# Autodesk Inventor assembly: HBLFSNF5-SEC_b
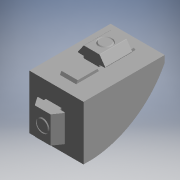
[picture p0: Inventor's stored thumbnail of the model, 180x180]
Saved by Autodesk Inventor 2017.3 (Build 213256000, 256)
## iProperties
Category: PARTsolutions
Company: MISUMI
Part Number: HBLFSNF5-SEC_b
Catalog Web Link: www.cadenas.de
Description: hblfsnf8_blacket-Tabbed Brackets - 1 Slots - HFS5 Series (Aluminum Extrusions 20, 25, 40 Square) - Reversal Tabbed Brackets (Depth 20mm)
Vendor: MISUMI
Document SubType Name: Assembly
Designer: partserver
Manufacturer: MISUMI
Mass: 6.66509 g
Surface Area: 56.4365 cm^2
Volume: 6.66509 cm^3
Density: 1 g/cm^3
Title: HBLFSNF5-SEC
Author: Cadenas PARTsolutions
Comments: Tabbed Brackets - 1 Slots - HFS5 Series (Aluminum Extrusions 20, 25, 40 Square) - Reversal Tabbed Brackets (Depth 20mm)
PSOL_IDENT_0: {$CADENAS_DATA\23d-libs\misumi\metric\38_al_extrusions_blackets\5\hblfsnf5_asmtab.prj},199 {VTYP=3D}
PSOL_IDENT_1: ,{STYP=ASSTAB},{NB=HBLFSNF5-SEC_b},{LINA=HBLFSNF5-SEC},{NN=hblfsnf8_blacket},{DATE=09.09.2019 15:28:
PSOL_IDENT_2: 10},{GEOMDATE=18.03.2016 03:17:17},{VERSION=},{LINEID=10},{WBVAR=ALT1,ALT2},{WBNUMERIC=}  {NB=HBLFSN
PSOL_IDENT_3: F5-SEC_b},{LINA=HBLFSNF5-SEC},{KT=DUMMY},{PN=HBLFSNF5-SEC},{TYPE=HBLFSNF5},{AS=HCBST5-12},{ASQ=2},{A
PSOL_IDENT_4: TN=HNTT5-5},{ATNQ=2},{ALT1=},{ALT2=-SEC},{ALT2ALG= '' , 'w/o Applicable Screws and Nuts Set' , '-SET'
PSOL_IDENT_5: , 'with SET (Applicable Screws and Nuts Set)' , '-SST' , 'with SST (Applicable Screws and Nuts Set(
PSOL_IDENT_6: Stainless Steel))' , '-SEU' , 'with SEU (Applicable Screws and Nuts Set(Pre-Assembly Insertion Sprin
PSOL_IDENT_7: g Nuts))' , '-SSU' , 'with SSU (Applicable Screws and Nuts Set(Pre-Assembly Insertion Spring Nuts St
PSOL_IDENT_8: ainless Steel))'  , '-SEP' , 'with SEP (Applicable Screws and Nuts Set(Post-Assembly Insertion Sprin
PSOL_IDENT_9: g Nuts))' , '-SSP' , 'with SSP (Applicable Screws and Nuts Set(Post-Assembly Insertion Spring Nuts S
PSOL_IDENT_10: tainless Steel))', '-SEC' , 'with SEC (Applicable Screws and Nuts Set(Washer Integrated Screws and N
PSOL_IDENT_11: uts))' },{SMAT=1010 Carbon Steel Equivalent},{SALT2=3},{NALT2=1},{M=5},{PPATH=hblfsnf5/hblfsnf5_asmt
PSOL_IDENT_12: pl.prj}
NB: HBLFSNF5-SEC_b
NN: hblfsnf8_blacket
NT: Tabbed Brackets - 1 Slots - HFS5 Series (Aluminum Extrusions 20, 25, 40 Square) - Reversal Tabbed Brackets (Depth 20mm)
NBSYN: $PN._b
LINA: HBLFSNF5-SEC
CATALOG: Misumi
PN: HBLFSNF5-SEC
TYPE: HBLFSNF5
AS: HCBST5-12
ASQ: 2
ATN: HNTT5-5
ATNQ: 2
ALT1: w/o C (Mounting Holes for Cover)
ALT2: with SEC (Applicable Screws and Nuts Set(Washer Integrated Screws and Nuts))
SUPPLIER: MISUMI
ARTICLENO: HBLFSNF5-SEC_b
BOMINFO: HBLFSNF5-SEC
CREATOR: CADENAS GmbH
## Documents named in this file (6)
- e:\temp\worker_16\temp\exporttempdir_5500_10_Vy7Sc\format_0\HBLFSNF5-SEC_b.iam
- e:\temp\worker_16\temp\exporttempdir_5500_10_Vy7Sc\format_0\HBLFSNF5-SEC_b.ipt
- e:\temp\worker_16\temp\exporttempdir_5500_10_Vy7Sc\format_0\HCBST5-12_s.ipt
- e:\temp\worker_16\temp\exporttempdir_5500_10_Vy7Sc\format_0\SPRING_WASHER5_1-9_2-1_3.ipt
- e:\temp\worker_16\temp\exporttempdir_5500_10_Vy7Sc\format_0\HCBST5w.ipt
- e:\temp\worker_16\temp\exporttempdir_5500_10_Vy7Sc\format_0\HNTT5-5.ipt
## Components (9 placed, 5 different names)
1. HBLFSNF5-SEC_b:1 — to_bolt1_XY@1 <-> to_body_XY@2, to_bolt1_Z@1 <-> to_body_Z@2, to_bolt1_YZ@1 <-> to_body_YZ@2, to_bolt2_XY@1 <-> to_body_XY@5, to_bolt2_Z@1 <-> to_body_Z@5, to_bolt2_YZ@1 <-> to_body_YZ@5, to_nut1_XY@1 <-> nut_XY@8, to_nut1_Z@1 <-> nut_Z@8, to_nut1_YZ@1 <-> nut_YZ@8, to_nut2_XY@1 <-> nut_XY@9, to_nut2_Z@1 <-> nut_Z@9, to_nut2_YZ@1 <-> nut_YZ@9
2. HCBST5-12_s:1 — to_bolt1_XY@1 <-> to_body_XY@2, to_bolt1_Z@1 <-> to_body_Z@2, to_bolt1_YZ@1 <-> to_body_YZ@2, bolt_to_spring_washer_XY@2 <-> to_bolt_XY@3, bolt_to_spring_washer_Z@2 <-> to_bolt_Z@3, bolt_to_spring_washer_YZ@2 <-> to_bolt_YZ@3, bolt_to_plane_washer_XY@2 <-> washer_to_bolt_XY@4, bolt_to_plane_washer_Z@2 <-> washer_to_bolt_Z@4, bolt_to_plane_washer_YZ@2 <-> washer_to_bolt_YZ@4
3. SPRING_WASHER5_1-9_2-1_3:1 — bolt_to_spring_washer_XY@2 <-> to_bolt_XY@3, bolt_to_spring_washer_Z@2 <-> to_bolt_Z@3, bolt_to_spring_washer_YZ@2 <-> to_bolt_YZ@3
4. HCBST5w:1 — bolt_to_plane_washer_XY@2 <-> washer_to_bolt_XY@4, bolt_to_plane_washer_Z@2 <-> washer_to_bolt_Z@4, bolt_to_plane_washer_YZ@2 <-> washer_to_bolt_YZ@4
5. HCBST5-12_s:2 — to_bolt2_XY@1 <-> to_body_XY@5, to_bolt2_Z@1 <-> to_body_Z@5, to_bolt2_YZ@1 <-> to_body_YZ@5, bolt_to_spring_washer_XY@5 <-> to_bolt_XY@6, bolt_to_spring_washer_Z@5 <-> to_bolt_Z@6, bolt_to_spring_washer_YZ@5 <-> to_bolt_YZ@6, bolt_to_plane_washer_XY@5 <-> washer_to_bolt_XY@7, bolt_to_plane_washer_Z@5 <-> washer_to_bolt_Z@7, bolt_to_plane_washer_YZ@5 <-> washer_to_bolt_YZ@7
6. SPRING_WASHER5_1-9_2-1_3:2 — bolt_to_spring_washer_XY@5 <-> to_bolt_XY@6, bolt_to_spring_washer_Z@5 <-> to_bolt_Z@6, bolt_to_spring_washer_YZ@5 <-> to_bolt_YZ@6
7. HCBST5w:2 — bolt_to_plane_washer_XY@5 <-> washer_to_bolt_XY@7, bolt_to_plane_washer_Z@5 <-> washer_to_bolt_Z@7, bolt_to_plane_washer_YZ@5 <-> washer_to_bolt_YZ@7
8. HNTT5-5:1 — to_nut1_XY@1 <-> nut_XY@8, to_nut1_Z@1 <-> nut_Z@8, to_nut1_YZ@1 <-> nut_YZ@8
9. HNTT5-5:2 — to_nut2_XY@1 <-> nut_XY@9, to_nut2_Z@1 <-> nut_Z@9, to_nut2_YZ@1 <-> nut_YZ@9
## Relationships (24: Mate 16, Angle 8)
- to_bolt1_XY@1 <-> to_body_XY@2 [Mate]: HBLFSNF5-SEC_b:1 ↔ HCBST5-12_s:1
- to_bolt1_Z@1 <-> to_body_Z@2 [Mate]: HBLFSNF5-SEC_b:1 ↔ HCBST5-12_s:1
- to_bolt1_YZ@1 <-> to_body_YZ@2 [Angle] (0 deg): HBLFSNF5-SEC_b:1 ↔ HCBST5-12_s:1
- bolt_to_spring_washer_XY@2 <-> to_bolt_XY@3 [Mate]: HCBST5-12_s:1 ↔ SPRING_WASHER5_1-9_2-1_3:1
- bolt_to_spring_washer_Z@2 <-> to_bolt_Z@3 [Mate]: HCBST5-12_s:1 ↔ SPRING_WASHER5_1-9_2-1_3:1
- bolt_to_spring_washer_YZ@2 <-> to_bolt_YZ@3 [Angle] (0 deg): HCBST5-12_s:1 ↔ SPRING_WASHER5_1-9_2-1_3:1
- bolt_to_plane_washer_XY@2 <-> washer_to_bolt_XY@4 [Mate]: HCBST5-12_s:1 ↔ HCBST5w:1
- bolt_to_plane_washer_Z@2 <-> washer_to_bolt_Z@4 [Mate]: HCBST5-12_s:1 ↔ HCBST5w:1
- bolt_to_plane_washer_YZ@2 <-> washer_to_bolt_YZ@4 [Angle] (0 deg): HCBST5-12_s:1 ↔ HCBST5w:1
- to_bolt2_XY@1 <-> to_body_XY@5 [Mate]: HBLFSNF5-SEC_b:1 ↔ HCBST5-12_s:2
- to_bolt2_Z@1 <-> to_body_Z@5 [Mate]: HBLFSNF5-SEC_b:1 ↔ HCBST5-12_s:2
- to_bolt2_YZ@1 <-> to_body_YZ@5 [Angle] (0 deg): HBLFSNF5-SEC_b:1 ↔ HCBST5-12_s:2
- bolt_to_spring_washer_XY@5 <-> to_bolt_XY@6 [Mate]: HCBST5-12_s:2 ↔ SPRING_WASHER5_1-9_2-1_3:2
- bolt_to_spring_washer_Z@5 <-> to_bolt_Z@6 [Mate]: HCBST5-12_s:2 ↔ SPRING_WASHER5_1-9_2-1_3:2
- bolt_to_spring_washer_YZ@5 <-> to_bolt_YZ@6 [Angle] (0 deg): HCBST5-12_s:2 ↔ SPRING_WASHER5_1-9_2-1_3:2
- bolt_to_plane_washer_XY@5 <-> washer_to_bolt_XY@7 [Mate]: HCBST5-12_s:2 ↔ HCBST5w:2
- bolt_to_plane_washer_Z@5 <-> washer_to_bolt_Z@7 [Mate]: HCBST5-12_s:2 ↔ HCBST5w:2
- bolt_to_plane_washer_YZ@5 <-> washer_to_bolt_YZ@7 [Angle] (0 deg): HCBST5-12_s:2 ↔ HCBST5w:2
- to_nut1_XY@1 <-> nut_XY@8 [Mate]: HBLFSNF5-SEC_b:1 ↔ HNTT5-5:1
- to_nut1_Z@1 <-> nut_Z@8 [Mate]: HBLFSNF5-SEC_b:1 ↔ HNTT5-5:1
- to_nut1_YZ@1 <-> nut_YZ@8 [Angle] (0 deg): HBLFSNF5-SEC_b:1 ↔ HNTT5-5:1
- to_nut2_XY@1 <-> nut_XY@9 [Mate]: HBLFSNF5-SEC_b:1 ↔ HNTT5-5:2
- to_nut2_Z@1 <-> nut_Z@9 [Mate]: HBLFSNF5-SEC_b:1 ↔ HNTT5-5:2
- to_nut2_YZ@1 <-> nut_YZ@9 [Angle] (0 deg): HBLFSNF5-SEC_b:1 ↔ HNTT5-5:2
